# Autodesk Inventor assembly: Assem4
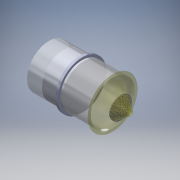
[picture p0: Inventor's stored thumbnail of the model, 180x180]
Saved by Autodesk Inventor 2017 (Build 210142000, 142)
## iProperties
Created: 2017-01-30
Part Number: Assem4
Document SubType Name: Assembly
Designer: XuZhiqing
Author: XuZhiqing
Sending System: SolidWorks 2015
Last Author: amirimah
Last Saved: 2017-01-30
## Documents named in this file (6)
- C:\Users\XuZhiqing\Desktop\Project01-CFD_the_sys\CAD-Mahtab filters\filter 01\Assem4.iam
- C:\Users\XuZhiqing\Desktop\Project01-CFD_the_sys\CAD-Mahtab filters\filter 01\Part1^Assem4.ipt
- C:\Users\XuZhiqing\Desktop\Project01-CFD_the_sys\CAD-Mahtab filters\filter 01\body1.ipt
- C:\Users\XuZhiqing\Desktop\Project01-CFD_the_sys\CAD-Mahtab filters\filter 01\safety valve filter.ipt
- C:\Users\XuZhiqing\Desktop\Project01-CFD_the_sys\CAD-Mahtab filters\filter 01\coneish.ipt
- C:\Users\XuZhiqing\Desktop\Project01-CFD_the_sys\CAD-Mahtab filters\filter 01\Part10.ipt
## Components (6 placed, 5 different names)
1. Part1^Assem4:1
2. body1:1 — Mate:1, Mate:2, Mate:3, Mate:4, Mate:5, Mate:7
3. safety valve filter:1 — Mate:4, Mate:6, Mate:7
4. body1:2 — Mate:5, Mate:6
5. coneish:1 — Mate:1, Mate:2
6. Part10:1 — Mate:3
## Relationships (7: Mate 7)
- Mate:1: body1:1 ↔ coneish:1
- Mate:2: body1:1 ↔ coneish:1
- Mate:3: body1:1 ↔ Part10:1
- Mate:4: body1:1 ↔ safety valve filter:1
- Mate:5: body1:1 ↔ body1:2
- Mate:6: safety valve filter:1 ↔ body1:2
- Mate:7: body1:1 ↔ safety valve filter:1
